# Autodesk Inventor assembly: 조립품1
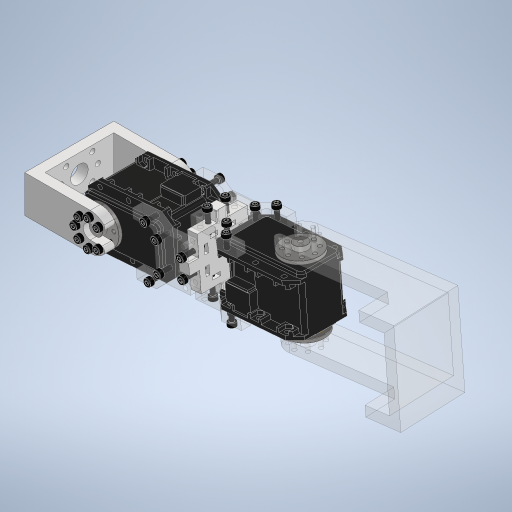
[picture p0: Inventor's stored thumbnail of the model, 512x512]
Saved by Autodesk Inventor 2024 (Build 280153000, 153)
## iProperties
Created: 2024-09-18
Part Number: 조립품1
Document SubType Name: Assembly
Designer: Eungang
Author: Eungang
## Documents named in this file (10)
- C:\Users\Eungang\Documents\Inventor\FIGHTING_ROBOT_FINAL\부품\Right_Arm\조립품1.iam
- C:\Users\Eungang\Documents\Inventor\FIGHTING_ROBOT_FINAL\부품\arm\arm_connect_3.ipt
- C:\Users\Eungang\Documents\Inventor\FIGHTING_ROBOT_FINAL\부품\arm\arm_connect_5.ipt
- C:\Users\Eungang\Documents\Inventor\FIGHTING_ROBOT_FINAL\부품\다이나믹셀\MX-28T_R.ipt
- C:\Users\Eungang\Documents\Inventor\FIGHTING_ROBOT_FINAL\부품\아이들러\28아이들러.iam
- C:\Users\Eungang\Documents\Inventor\FIGHTING_ROBOT_FINAL\부품\혼\28Horn.ipt
- C:\Users\Eungang\Documents\Inventor\FIGHTING_ROBOT_FINAL\부품\Bolt_Washer_Nut\CSH-ST-M2_5-8_203.ipt
- C:\Users\Eungang\Documents\Inventor\FIGHTING_ROBOT_FINAL\부품\Bolt_Washer_Nut\Arm_bolt_set_2_5_8 x 6.iam
- C:\Users\Eungang\Documents\Inventor\FIGHTING_ROBOT_FINAL\부품\Bolt_Washer_Nut\arm_motor_connect.ipt
- C:\Users\Eungang\Documents\Inventor\Fighting_Robot\부품56.ipt
## Components (31 placed, 9 different names)
1. arm_connect_3:1 — 메이트:1, 삽입:8, 삽입:9, 삽입:10, 삽입:11, 삽입:12, 삽입:13, 삽입:14, 삽입:15, 삽입:16, 삽입:17, 삽입:18, 삽입:19, 삽입:20, 삽입:21, 삽입:22
2. arm_connect_5:1 — 삽입:4, 삽입:5, 삽입:23, 삽입:24
3. MX-28T_R:1 — 삽입:1, 삽입:2, 삽입:4, 삽입:5, 삽입:6, 삽입:7, 플러쉬:1, 플러쉬:2
4. 28아이들러:1 [sub-assembly] — 삽입:2
5. 28Horn:1 — 삽입:1, 삽입:8
6. arm_connect_5:2 — 삽입:6, 삽입:7, 삽입:25, 삽입:26
7. CSH-ST-M2_5-8_203:1 — 삽입:16
8. CSH-ST-M2_5-8_203:2 — 삽입:11
9. CSH-ST-M2_5-8_203:3 — 삽입:13
10. CSH-ST-M2_5-8_203:4 — 삽입:15
11. CSH-ST-M2_5-8_203:5 — 삽입:14
12. CSH-ST-M2_5-8_203:6 — 삽입:12
13. CSH-ST-M2_5-8_203:7 — 삽입:9
14. CSH-ST-M2_5-8_203:8 — 삽입:10
15. CSH-ST-M2_5-8_203:9 — 삽입:19
16. CSH-ST-M2_5-8_203:10 — 삽입:18
17. CSH-ST-M2_5-8_203:11 — 삽입:17
18. CSH-ST-M2_5-8_203:12 — 삽입:20
19. CSH-ST-M2_5-8_203:13 — 삽입:21
20. CSH-ST-M2_5-8_203:14 — 삽입:22
21. Arm_bolt_set_2_5_8 x 6:1 [sub-assembly] — 삽입:23, 삽입:24
22. Arm_bolt_set_2_5_8 x 6:2 [sub-assembly] — 삽입:25, 삽입:26
23. arm_connect_5:3 — 삽입:40, 삽입:41
24. MX-28T_R:2 — 플러쉬:1, 플러쉬:2
25. 28아이들러:2 [sub-assembly] — 삽입:38
26. 28Horn:2 — 삽입:37, 삽입:39
27. arm_connect_5:4
28. Arm_bolt_set_2_5_8 x 6:3 [sub-assembly]
29. Arm_bolt_set_2_5_8 x 6:4 [sub-assembly]
30. arm_motor_connect:1 — 삽입:40, 삽입:41
31. 부품56:1 — 삽입:37, 삽입:38, 삽입:39
## Relationships (43: Insert 40, Flush 2, Mate 1)
- 메이트:1 [Mate]: arm_connect_3:1
- 삽입:1 [Insert] (0.75 mm): MX-28T_R:1 ↔ 28Horn:1
- 삽입:2 [Insert] (0.75 mm): MX-28T_R:1 ↔ 28아이들러:1
- 삽입:4 [Insert]: arm_connect_5:1 ↔ MX-28T_R:1
- 삽입:5 [Insert]: arm_connect_5:1 ↔ MX-28T_R:1
- 삽입:6 [Insert]: MX-28T_R:1 ↔ arm_connect_5:2
- 삽입:7 [Insert]: MX-28T_R:1 ↔ arm_connect_5:2
- 삽입:8 [Insert]: arm_connect_3:1 ↔ 28Horn:1
- 삽입:9 [Insert]: arm_connect_3:1 ↔ CSH-ST-M2_5-8_203:7
- 삽입:10 [Insert]: arm_connect_3:1 ↔ CSH-ST-M2_5-8_203:8
- 삽입:11 [Insert]: arm_connect_3:1 ↔ CSH-ST-M2_5-8_203:2
- 삽입:12 [Insert]: arm_connect_3:1 ↔ CSH-ST-M2_5-8_203:6
- 삽입:13 [Insert]: arm_connect_3:1 ↔ CSH-ST-M2_5-8_203:3
- 삽입:14 [Insert]: arm_connect_3:1 ↔ CSH-ST-M2_5-8_203:5
- 삽입:15 [Insert]: arm_connect_3:1 ↔ CSH-ST-M2_5-8_203:4
- 삽입:16 [Insert]: arm_connect_3:1 ↔ CSH-ST-M2_5-8_203:1
- 삽입:17 [Insert]: arm_connect_3:1 ↔ CSH-ST-M2_5-8_203:11
- 삽입:18 [Insert]: arm_connect_3:1 ↔ CSH-ST-M2_5-8_203:10
- 삽입:19 [Insert]: arm_connect_3:1 ↔ CSH-ST-M2_5-8_203:9
- 삽입:20 [Insert]: arm_connect_3:1 ↔ CSH-ST-M2_5-8_203:12
- 삽입:21 [Insert]: arm_connect_3:1 ↔ CSH-ST-M2_5-8_203:13
- 삽입:22 [Insert]: arm_connect_3:1 ↔ CSH-ST-M2_5-8_203:14
- 삽입:23 [Insert]: arm_connect_5:1 ↔ Arm_bolt_set_2_5_8 x 6:1
- 삽입:24 [Insert]: arm_connect_5:1 ↔ Arm_bolt_set_2_5_8 x 6:1
- 삽입:25 [Insert]: arm_connect_5:2 ↔ Arm_bolt_set_2_5_8 x 6:2
- 삽입:26 [Insert]: arm_connect_5:2 ↔ Arm_bolt_set_2_5_8 x 6:2
- [Insert] (0.75 mm): MX-28T_R:2 ↔ 28Horn:2
- [Insert] (0.75 mm): MX-28T_R:2 ↔ 28아이들러:2
- [Insert]: arm_connect_5:3 ↔ MX-28T_R:2
- [Insert]: arm_connect_5:3 ↔ MX-28T_R:2
- [Insert]: MX-28T_R:2 ↔ arm_connect_5:4
- [Insert]: MX-28T_R:2 ↔ arm_connect_5:4
- [Insert]: arm_connect_5:3 ↔ Arm_bolt_set_2_5_8 x 6:3
- [Insert]: arm_connect_5:3 ↔ Arm_bolt_set_2_5_8 x 6:3
- [Insert]: arm_connect_5:4 ↔ Arm_bolt_set_2_5_8 x 6:4
- [Insert]: arm_connect_5:4 ↔ Arm_bolt_set_2_5_8 x 6:4
- 플러쉬:1 [Flush]: MX-28T_R:1 ↔ MX-28T_R:2
- 플러쉬:2 [Flush]: MX-28T_R:1 ↔ MX-28T_R:2
- 삽입:37 [Insert] (0.1 mm): 28Horn:2 ↔ 부품56:1
- 삽입:38 [Insert] (0.1 mm): 28아이들러:2 ↔ 부품56:1
- 삽입:39 [Insert] (0.1 mm): 28Horn:2 ↔ 부품56:1
- 삽입:40 [Insert] (0.1 mm): arm_connect_5:3 ↔ arm_motor_connect:1
- 삽입:41 [Insert] (0.1 mm): arm_connect_5:3 ↔ arm_motor_connect:1
## Named parameters: d29_d1 = 0.75 mm, d30_d2 = 0.75 mm, d31_d4 = 0 mm, d32_d5 = 0 mm, d33_d6 = 0 mm, d34_d7 = 0 mm, d35_d25 = 0 mm, d36_d26 = 0 mm, d37_d27 = 0 mm, d38_d28 = 0 mm
